# Autodesk Inventor assembly: RailBlock
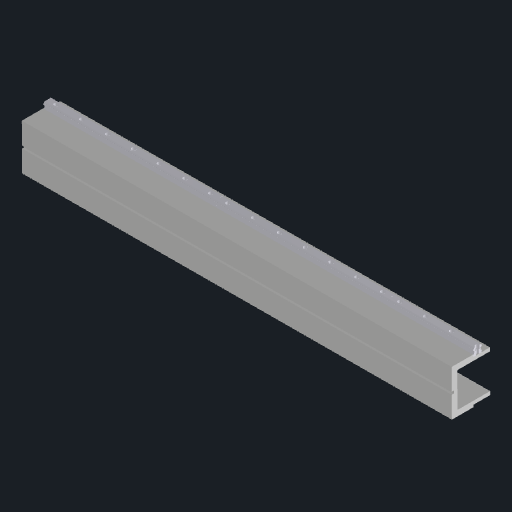
[picture p0: Inventor's stored thumbnail of the model, 512x512]
Saved by Autodesk Inventor 2024 (Build 280153000, 153)
## iProperties
Created: 2023-03-08
Part Number: RailBlock
Document SubType Name: Assembly
Designer: KirikDK
Mass: 2962.42 g
Surface Area: 9629.04 cm^2
Volume: 2962.42 cm^3
Density: 1 g/cm^3
Author: KirikDK
## Documents named in this file (6)
- C:\Users\KirikDK\Documents\Stanok2023\RailBlock.iam
- C:\Users\KirikDK\Documents\Stanok2023\Ugolok1000.ipt
- C:\Users\KirikDK\Documents\Stanok2023\Plate8_80_1000.ipt
- C:\Users\KirikDK\Documents\Stanok2023\Stenki.ipt
- C:\Users\KirikDK\Documents\Stanok2023\mgn20_1000.ipt
- C:\Users\KirikDK\Documents\Stanok2023\InsidePereborka.ipt
## Components (11 placed, 5 different names)
1. Ugolok1000:1 — Совмещение:5, Заподлицо:7, Совмещение:6, Заподлицо:9, Заподлицо:10, Заподлицо:13, Заподлицо:15, Заподлицо:17
2. Ugolok1000:2 — Совмещение:3, Совмещение:4, Совмещение:15, Заподлицо:18, Заподлицо:19
3. Plate8_80_1000:1 — Заподлицо:2, Совмещение:2, Заподлицо:4, Совмещение:3, Совмещение:4, Заподлицо:7, Совмещение:6, Совмещение:13, Совмещение:14, Заподлицо:19
4. Stenki:1 — Заподлицо:2, Совмещение:2, Заподлицо:4, Совмещение:5, Заподлицо:8, Совмещение:7, Заподлицо:11, Заподлицо:12, Заподлицо:14, Заподлицо:16, Совмещение:12
5. mgn20_1000:1 — Заподлицо:8, Заподлицо:9, Совмещение:7, Совмещение:8
6. mgn20_1000:2 — Заподлицо:10, Заподлицо:11, Совмещение:8, Совмещение:9
7. mgn20_1000:3 — Заподлицо:12, Совмещение:9, Заподлицо:13, Совмещение:10
8. mgn20_1000:4 — Заподлицо:14, Совмещение:10, Заподлицо:15, Совмещение:11
9. mgn20_1000:5 — Совмещение:11, Заподлицо:16, Заподлицо:17
10. InsidePereborka:1 — Совмещение:12, Совмещение:13
11. Stenki:2 — Совмещение:14, Совмещение:15, Заподлицо:18
## Relationships (29: Flush 15, Mate 14)
- Заподлицо:2 [Flush]: Plate8_80_1000:1 ↔ Stenki:1
- Совмещение:2 [Mate]: Plate8_80_1000:1 ↔ Stenki:1
- Заподлицо:4 [Flush]: Plate8_80_1000:1 ↔ Stenki:1
- Совмещение:3 [Mate]: Ugolok1000:2 ↔ Plate8_80_1000:1
- Совмещение:4 [Mate]: Ugolok1000:2 ↔ Plate8_80_1000:1
- Совмещение:5 [Mate]: Ugolok1000:1 ↔ Stenki:1
- Заподлицо:7 [Flush]: Ugolok1000:1 ↔ Plate8_80_1000:1
- Совмещение:6 [Mate]: Ugolok1000:1 ↔ Plate8_80_1000:1
- Заподлицо:8 [Flush]: Stenki:1 ↔ mgn20_1000:1
- Заподлицо:9 [Flush]: Ugolok1000:1 ↔ mgn20_1000:1
- Совмещение:7 [Mate]: Stenki:1 ↔ mgn20_1000:1
- Заподлицо:10 [Flush]: Ugolok1000:1 ↔ mgn20_1000:2
- Заподлицо:11 [Flush]: Stenki:1 ↔ mgn20_1000:2
- Совмещение:8 [Mate]: mgn20_1000:1 ↔ mgn20_1000:2
- Заподлицо:12 [Flush]: Stenki:1 ↔ mgn20_1000:3
- Совмещение:9 [Mate]: mgn20_1000:2 ↔ mgn20_1000:3
- Заподлицо:13 [Flush]: Ugolok1000:1 ↔ mgn20_1000:3
- Заподлицо:14 [Flush]: Stenki:1 ↔ mgn20_1000:4
- Совмещение:10 [Mate]: mgn20_1000:3 ↔ mgn20_1000:4
- Заподлицо:15 [Flush]: Ugolok1000:1 ↔ mgn20_1000:4
- Совмещение:11 [Mate]: mgn20_1000:4 ↔ mgn20_1000:5
- Заподлицо:16 [Flush]: Stenki:1 ↔ mgn20_1000:5
- Заподлицо:17 [Flush]: Ugolok1000:1 ↔ mgn20_1000:5
- Совмещение:12 [Mate]: Stenki:1 ↔ InsidePereborka:1
- Совмещение:13 [Mate]: Plate8_80_1000:1 ↔ InsidePereborka:1
- Совмещение:14 [Mate]: Plate8_80_1000:1 ↔ Stenki:2
- Совмещение:15 [Mate]: Ugolok1000:2 ↔ Stenki:2
- Заподлицо:18 [Flush]: Ugolok1000:2 ↔ Stenki:2
- Заподлицо:19 [Flush]: Ugolok1000:2 ↔ Plate8_80_1000:1
